# Autodesk Inventor assembly: SKF_NKX 12 Z
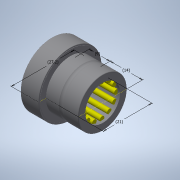
[picture p0: Inventor's stored thumbnail of the model, 180x180]
Saved by Autodesk Inventor 2022 (Build 260153000, 153)
## iProperties
Created: 2022-07-21
Part Number: SKF_NKX 12 Z
Catalog Web Link: www.cadenas.de
Description: BVN_002_003-Needle roller / thrust rolling bearings
Vendor: SKF
Document SubType Name: Assembly
Designer: psAdmin
Manufacturer: SKF
Mass: 40 g
Surface Area: 69.2571 cm^2
Volume: 6.12695 cm^3
Density: 6.52853 g/cm^3
Category: PARTsolutions
Company: SKF
PSOL_IDENT_0: {$CADENAS_DATA/23d-libs/skf/bearings_units_and_housings/roller_bearings/needle_roller_bearings/bvn_0
PSOL_IDENT_1: 02_003.prj},172 {VTYP=3D},{NB=SKF_NKX 12 Z},{LINA=SKF_NKX 12 Z},{NN=BVN_002_003},{DATE=08.07.2022 10
PSOL_IDENT_2: :25:50},{GEOMDATE=06.12.2021 10:15:46},{VERSION=},{LINEID=10220},{WBVAR=},{WBNUMERIC=}  {NB=SKF_NKX
PSOL_IDENT_3: 12 Z},{LINA=SKF_NKX 12 Z},{KT=DUMMY},{DESIGNATION=NKX 12 Z},{DESIGN=comb_nkxz},{SB=ball},{DESIGNZ=1}
PSOL_IDENT_4: ,{F=12},{FW=12},{FALG=12.000},{D=21.000},{C=23.000},{C1=9},{C2=6.5},{DD=12.000},{D1=26.1},{D2=27.200
PSOL_IDENT_5: },{R12=0.300},{PITCH=14.000},{PITCHA=19.000},{ALPHAA=0.000},{DW=2.000},{DWA=4.762},{LW=12.800},{LWA=
PSOL_IDENT_6: 0.000},{DA=21.700},{LOAD1=9.130},{LOAD2=12.000},{LOAD3=10.400},{LOAD4=16.600},{LOAD5=1.430},{LOAD6=0
PSOL_IDENT_7: .620},{LOADA=0.0},{SPEED1=9000},{SPEED2=7500},{Z=13.000},{ZA=11.000},{II=1.000},{IIA=0.000},{MASS=0.
PSOL_IDENT_8: 040},{C3=0.000},{C1A=9},{DAMAX=},{SPEED1X=},{RAMAX=0.3},{IIX=},{LWX=},{LOAD4X=},{SPEED2X=},{ZX=11},{
PSOL_IDENT_9: LOAD6X=},{ALPHAX=},{LOAD3X=},{ALPHA=90},{RBMAX=0.3},{DWXX=},{PITCHXX=},{DI=9},{DDAMIN=21.7},{DWX=4.7
PSOL_IDENT_10: 62},{C1X=6.5},{ZXX=},{LOADAX=},{POPULAR=Yes},{PITCHX=19},{BI=16},{D1ALG=26.100},{C2ALG=6.500},{PITCH
PSOL_IDENT_11: XXA=0.000},{LWXA=0.000},{DWXXA=0.000},{DIA=9.000}
NB: SKF_NKX 12 Z
NN: BVN_002_003
NT: Needle roller / thrust rolling bearings
NBSYN: SKF_$DESIGNATION.
LINA: SKF_NKX 12 Z
CATALOG: SKF
DESIGNATION: NKX 12 Z
F: 12
D: 21
C: 23
C1: 9
C2: 6.5
DD: 12
D2: 27.2
R12: 0.3
LOAD1: 9.13
LOAD2: 12
LOAD3: 10.4
LOAD4: 16.6
LOAD5: 1.43
LOAD6: 0.62
LOADA: 0
SPEED1: 9000
SPEED2: 7500
MASS: 0.04
SUPPLIER: SKF
ARTICLENO: SKF_NKX 12 Z
BOMINFO: SKF_NKX 12 Z
CREATOR: CADENAS GmbH
NKX_12_AxialPart_Width: 9,000 mm
NKX_12_RadialPart_Width: 14,000 mm
NKX_12_RadialPart_Diameter: 21,000 mm
NKX_12_maxOuterDia: 27,200 mm
Title: SKF_NKX 12 Z
Author: Cadenas PARTsolutions
Comments: Needle roller / thrust rolling bearings
## Documents named in this file (4)
- C:\Users\alexw\Documents\Inventor\Projects\03_CurrentProjects\MasterThesis\Parallelsystem_DaVinci_CAD\Downloads\SKF_NKX 12 Z\SKF_NKX 12 Z.iam
- C:\Users\alexw\Documents\Inventor\Projects\03_CurrentProjects\MasterThesis\Parallelsystem_DaVinci_CAD\Downloads\SKF_NKX 12 Z\SKF_NKX 12 Z_PART1.ipt
- C:\Users\alexw\Documents\Inventor\Projects\03_CurrentProjects\MasterThesis\Parallelsystem_DaVinci_CAD\Downloads\SKF_NKX 12 Z\SKF_NKX 12 Z_PART2.ipt
- C:\Users\alexw\Documents\Inventor\Projects\03_CurrentProjects\MasterThesis\Parallelsystem_DaVinci_CAD\Downloads\SKF_NKX 12 Z\SKF_NKX 12 Z_PART3.ipt
## Components (27 placed, 3 different names)
1. SKF_NKX 12 Z_PART1:1
2. SKF_NKX 12 Z_PART2:1
3. SKF_NKX 12 Z_PART2:2
4. SKF_NKX 12 Z_PART2:3
5. SKF_NKX 12 Z_PART2:4
6. SKF_NKX 12 Z_PART2:5
7. SKF_NKX 12 Z_PART2:6
8. SKF_NKX 12 Z_PART2:7
9. SKF_NKX 12 Z_PART2:8
10. SKF_NKX 12 Z_PART2:9
11. SKF_NKX 12 Z_PART2:10
12. SKF_NKX 12 Z_PART2:11
13. SKF_NKX 12 Z_PART2:12
14. SKF_NKX 12 Z_PART2:13
15. SKF_NKX 12 Z_PART3:1
16. SKF_NKX 12 Z_PART3:2
17. SKF_NKX 12 Z_PART3:3
18. SKF_NKX 12 Z_PART3:4
19. SKF_NKX 12 Z_PART3:5
20. SKF_NKX 12 Z_PART3:6
21. SKF_NKX 12 Z_PART3:7
22. SKF_NKX 12 Z_PART3:8
23. SKF_NKX 12 Z_PART3:9
24. SKF_NKX 12 Z_PART3:10
25. SKF_NKX 12 Z_PART3:11
26. SKF_NKX 12 Z_PART3:12
27. SKF_NKX 12 Z_PART3:13
## Named parameters: NKX_12_AxialPart_Width = 9 mm, NKX_12_RadialPart_Width = 14 mm, NKX_12_RadialPart_Diameter = 21 mm, NKX_12_maxOuterDia = 27.2 mm
